(part 1 of 2)
# Autodesk Inventor assembly: Additional_Building
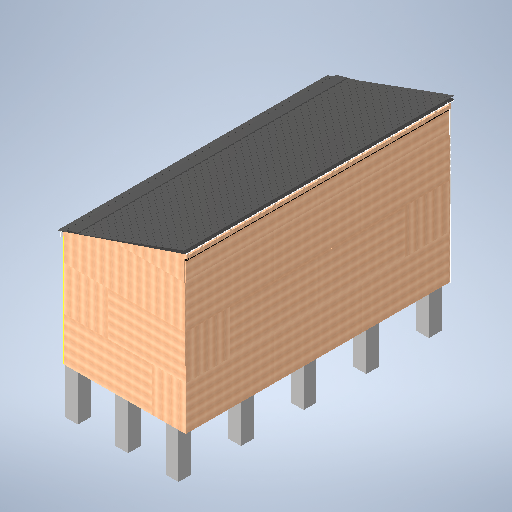
[picture p0: Inventor's stored thumbnail of the model, 512x512]
Saved by Autodesk Inventor 2025 (Build 290162010, 162A)
## iProperties
Created: 2024-08-02
Part Number: Additional_Building
Document SubType Name: Assembly
Designer: Tom
Author: Tom
## Documents named in this file (79)
- C:\Users\Tom\Documents\Inventor\Mobility\Additional_Building\Additional_Building.iam
- C:\Users\Tom\Documents\Inventor\Mobility\Additional_Building\Grid_Of_Piers.iam
- C:\Users\Tom\Documents\Inventor\Mobility\Additional_Building\Floor_System.iam
- C:\Users\Tom\Documents\Inventor\Mobility\Additional_Building\Framing_For_First_Floor.iam
- C:\Users\Tom\Documents\Inventor\Mobility\Additional_Building\Truss.iam
- C:\Users\Tom\Documents\Inventor\Mobility\Additional_Building\OSB_For_Walls_With_Dimensions_48_x_96_Inches.ipt
- C:\Users\Tom\Documents\Inventor\Mobility\Additional_Building\OSB_For_Walls_With_Dimensions_48_x_48_Inches.ipt
- C:\Users\Tom\Documents\Inventor\Mobility\Additional_Building\OSB_For_Roof_With_Dimensions_48_x_96.ipt
- C:\Users\Tom\Documents\Inventor\Mobility\Additional_Building\OSB_For_Walls_With_Dimensions_25.5_x_96_Inches.ipt
- C:\Users\Tom\Documents\Inventor\Mobility\Additional_Building\Subfascia_With_Dimensions_4.023_x_13.75_Inches.ipt
- C:\Users\Tom\Documents\Inventor\Mobility\Additional_Building\Subfascia_With_Dimensions_4.023_x_14.5_Inches.ipt
- C:\Users\Tom\Documents\Inventor\Mobility\Additional_Building\DensGlass_With_Dimensions_36.5_x_48_Inches.ipt
- C:\Users\Tom\Documents\Inventor\Mobility\Additional_Building\DensGlass_With_Dimensions_48_x_96_Inches.ipt
- C:\Users\Tom\Documents\Inventor\Mobility\Additional_Building\DensGlass_With_Dimensions_48_x_84.5_Inches.ipt
- C:\Users\Tom\Documents\Inventor\Mobility\Additional_Building\DensGlass_With_Dimensions_12_x_60.75_Inches.ipt
- C:\Users\Tom\Documents\Inventor\Mobility\Additional_Building\DensGlass_With_Dimensions_25.5_x_36.5_Inches.ipt
- C:\Users\Tom\Documents\Inventor\Mobility\Additional_Building\DensGlass_With_Dimensions_25.5_x_96_Inches.ipt
- C:\Users\Tom\Documents\Inventor\Mobility\Additional_Building\Siding_For_Back_Wall.iam
- C:\Users\Tom\Documents\Inventor\Mobility\Additional_Building\Fascia_For_Back.ipt
- C:\Users\Tom\Documents\Inventor\Mobility\Additional_Building\OSB_For_Side_And_Back.ipt
- C:\Users\Tom\Documents\Inventor\Mobility\Additional_Building\OSB_For_Roof_With_Dimensions_48_x_48.ipt
- C:\Users\Tom\Documents\Inventor\Mobility\Additional_Building\OSB_For_Roof_With_Dimensions_47.416_x_96.ipt
- C:\Users\Tom\Documents\Inventor\Mobility\Additional_Building\Stud_With_Height_4.254_Inches.ipt
- C:\Users\Tom\Documents\Inventor\Mobility\Additional_Building\Stud_With_Height_9.593_Inches.ipt
- C:\Users\Tom\Documents\Inventor\Mobility\Additional_Building\Stud_With_Height_14.931_Inches.ipt
- C:\Users\Tom\Documents\Inventor\Mobility\Additional_Building\Stud_With_Height_20.270_Inches.ipt
- C:\Users\Tom\Documents\Inventor\Mobility\Additional_Building\Stud_With_Height_25.608_Inches.ipt
- C:\Users\Tom\Documents\Inventor\Mobility\Additional_Building\Stud_With_Height_30.947_Inches.ipt
- C:\Users\Tom\Documents\Inventor\Mobility\Additional_Building\Stud_With_Height_36.285_Inches.ipt
- C:\Users\Tom\Documents\Inventor\Mobility\Additional_Building\Stud_With_Height_39.580_Inches.ipt
- C:\Users\Tom\Documents\Inventor\Mobility\Additional_Building\Stud_With_Height_41.707_Inches_And_Cut.ipt
- C:\Users\Tom\Documents\Inventor\Mobility\Additional_Building\Stud_With_Height_41.707_Inches.ipt
- C:\Users\Tom\Documents\Inventor\Mobility\Additional_Building\Support_For_Ceiling.ipt
- C:\Users\Tom\Documents\Inventor\Mobility\Additional_Building\OSB_For_Side_And_Front.ipt
- C:\Users\Tom\Documents\Inventor\Mobility\Additional_Building\OSB_For_Side_And_Top.ipt
- C:\Users\Tom\Documents\Inventor\Mobility\Additional_Building\Subfascia_With_Dimensions_3.725_x_13.75_Inches.ipt
- C:\Users\Tom\Documents\Inventor\Mobility\Additional_Building\Subfascia_With_Dimensions_3.725_x_14.5_Inches.ipt
- C:\Users\Tom\Documents\Inventor\Mobility\Additional_Building\OSB_For_Walls_With_Dimensions_21.107_x_48_Inches.ipt
- C:\Users\Tom\Documents\Inventor\Mobility\Additional_Building\OSB_For_Walls_With_Dimensions_21.107_x_96_Inches.ipt
- C:\Users\Tom\Documents\Inventor\Mobility\Additional_Building\Siding_For_Front_Wall.iam
- C:\Users\Tom\Documents\Inventor\Mobility\Additional_Building\Fascia_For_Front.ipt
- C:\Users\Tom\Documents\Inventor\Mobility\Additional_Building\OSB_For_Walls_With_Dimensions_48_x_85_Inches.ipt
- C:\Users\Tom\Documents\Inventor\Mobility\Additional_Building\OSB_For_Walls_With_Dimensions_37_x_48_Inches.ipt
- C:\Users\Tom\Documents\Inventor\Mobility\Additional_Building\Fascia_For_Side.ipt
- C:\Users\Tom\Documents\Inventor\Mobility\Additional_Building\Drip_Edge_For_Back.ipt
- C:\Users\Tom\Documents\Inventor\Mobility\Additional_Building\OSB_For_Rear_Roof.ipt
- C:\Users\Tom\Documents\Inventor\Mobility\Additional_Building\Siding_For_Left_Wall.iam
- C:\Users\Tom\Documents\Inventor\Mobility\Additional_Building\Siding_For_Right_Wall.iam
- C:\Users\Tom\Documents\Inventor\Mobility\Additional_Building\Drip_Edge_For_Side.ipt
- C:\Users\Tom\Documents\Inventor\Mobility\Additional_Building\Underlayment_For_Side.ipt
- C:\Users\Tom\Documents\Inventor\Mobility\Additional_Building\Underlayment_For_Front.ipt
- C:\Users\Tom\Documents\Inventor\Mobility\Additional_Building\Starter_Shingle_With_Dimensions_6.5_x_38_Inches.ipt
- C:\Users\Tom\Documents\Inventor\Mobility\Additional_Building\Leak_Barrier.ipt
- C:\Users\Tom\Documents\Inventor\Mobility\Additional_Building\Underlayment_For_Roof_With_Width_48_Inches.ipt
- C:\Users\Tom\Documents\Inventor\Mobility\Additional_Building\Underlayment_For_Roof_With_Width_19.157_Inches.ipt
- C:\Users\Tom\Documents\Inventor\Mobility\Additional_Building\Drip_Edge_For_Front.ipt
- C:\Users\Tom\Documents\Inventor\Mobility\Additional_Building\Starter_Shingle_With_Dimensions_6.5_x_35_Inches.ipt
- C:\Users\Tom\Documents\Inventor\Mobility\Additional_Building\Starter_Shingle_With_Dimensions_6.5_x_32.075_Inches.ipt
- C:\Users\Tom\Documents\Inventor\Mobility\Additional_Building\Starter_Shingle_With_Dimensions_6.5_x_29.875_Inches.ipt
- C:\Users\Tom\Documents\Inventor\Mobility\Additional_Building\Shingle_With_Dimensions_13.25_x_39.375_Inches.ipt
- C:\Users\Tom\Documents\Inventor\Mobility\Additional_Building\Shingle_With_Dimensions_13.25_x_19.45_Inches.ipt
- C:\Users\Tom\Documents\Inventor\Mobility\Additional_Building\Shingle_With_Dimensions_13.25_x_25.45_Inches.ipt
- C:\Users\Tom\Documents\Inventor\Mobility\Additional_Building\Bottom_Of_End_Cap_Of_Intake_Vent.ipt
- C:\Users\Tom\Documents\Inventor\Mobility\Additional_Building\Intake_Vent.ipt
- C:\Users\Tom\Documents\Inventor\Mobility\Additional_Building\Side_Of_End_Cap_For_Intake_Vent.ipt
- C:\Users\Tom\Documents\Inventor\Mobility\Additional_Building\First_Shingle_Over_Intake_Vent_With_Length_28.375_Inches.ipt
- C:\Users\Tom\Documents\Inventor\Mobility\Additional_Building\First_Shingle_Over_Intake_Vent_With_Length_39.375_Inches.ipt
- C:\Users\Tom\Documents\Inventor\Mobility\Additional_Building\First_Shingle_Over_Intake_Vent_With_Length_30.45_Inches.ipt
- C:\Users\Tom\Documents\Inventor\Mobility\Additional_Building\Second_Shingle_Over_Intake_Vent_With_Length_22.375_Inches.ipt
- C:\Users\Tom\Documents\Inventor\Mobility\Additional_Building\Second_Shingle_Over_Intake_Vent_With_Length_39.375_Inches.ipt
- C:\Users\Tom\Documents\Inventor\Mobility\Additional_Building\Second_Shingle_Over_Intake_Vent_With_Length_36.45_Inches.ipt
- C:\Users\Tom\Documents\Inventor\Mobility\Additional_Building\Third_Shingle_Over_Intake_Vent_With_Length_39.375_Inches.ipt
- C:\Users\Tom\Documents\Inventor\Mobility\Additional_Building\Third_Shingle_Over_Intake_Vent_With_Length_19.45_Inches.ipt
- C:\Users\Tom\Documents\Inventor\Mobility\Additional_Building\Shingle_With_Dimensions_13.25_x_33.375_Inches.ipt
- C:\Users\Tom\Documents\Inventor\Mobility\Additional_Building\Shingle_With_Dimensions_13.25_x_28.375_Inches.ipt
- C:\Users\Tom\Documents\Inventor\Mobility\Additional_Building\Shingle_With_Dimensions_13.25_x_30.45_Inches.ipt
- C:\Users\Tom\Documents\Inventor\Mobility\Additional_Building\Shingle_With_Dimensions_13.25_x_22.375_Inches.ipt
- C:\Users\Tom\Documents\Inventor\Mobility\Additional_Building\Shingle_With_Dimensions_13.25_x_36.45_Inches.ipt
- C:\Users\Tom\Documents\Inventor\Mobility\Additional_Building\Soffit_Strip_Vent.ipt
## Components (417 placed, 78 different names)
1. Grid_Of_Piers:1 [sub-assembly] — Mate:1, Flush:1, Mate:2
2. Floor_System:1 [sub-assembly] — Mate:1, Flush:1, Mate:2, Mate:3, Flush:2, Flush:3, Flush:15, Flush:16, Flush:29, Flush:30, Flush:31, Flush:33
3. Framing_For_First_Floor:1 [sub-assembly] — Mate:3, Flush:2, Flush:3, Flush:4, Flush:5, Mate:4, Flush:7, Mate:5, Mate:9, Mate:10, Flush:17, Mate:12, Mate:15, Mate:18, Mate:68, Flush:48, Flush:49, Mate:69, Flush:50, Flush:51, Mate:70, Flush:52, Flush:53, Mate:71, Flush:54, Flush:55, Mate:72, Flush:56, Flush:57, Mate:73, Flush:58, Flush:59, Mate:74, Flush:60, Flush:61, Mate:75, Flush:62, Flush:63, Mate:76, Flush:64, Mate:78, Mate:90, Mate:113, Mate:116, Mate:119, Mate:121
4. Subfascia_With_Dimensions_4.023_x_13.75_Inches:1 — Mate:21, Flush:22, Flush:23
5. Subfascia_With_Dimensions_4.023_x_13.75_Inches:2 — Flush:26, Mate:23, Flush:27, Flush:39
6. DensGlass_With_Dimensions_36.5_x_48_Inches:1 — Mate:24, Flush:28, Flush:29, Mate:26
7. DensGlass_With_Dimensions_36.5_x_48_Inches:2 — Mate:27, Mate:28, Flush:31
8. DensGlass_With_Dimensions_48_x_84.5_Inches:1 — Mate:29, Flush:32, Mate:30, Mate:32, Mate:38, Mate:41, Mate:44
9. DensGlass_With_Dimensions_48_x_96_Inches:3 — Mate:31, Mate:32, Mate:33, Mate:35
10. DensGlass_With_Dimensions_48_x_84.5_Inches:2 — Mate:34, Mate:35, Mate:36, Mate:47
11. DensGlass_With_Dimensions_25.5_x_36.5_Inches:1 — Mate:39, Mate:40, Mate:41, Mate:43
12. DensGlass_With_Dimensions_25.5_x_36.5_Inches:2 — Mate:45, Mate:46, Mate:47
13. Siding_For_Back_Wall:1 [sub-assembly] — Mate:48, Flush:34, Flush:35, Flush:158
14. Underlayment_For_Front:1 — Mate:146, Flush:126, Mate:147
15. Siding_For_Front_Wall:1 [sub-assembly] — Flush:93, Flush:94, Mate:108
16. Underlayment_For_Side:1 — Flush:122, Flush:157
17. Siding_For_Left_Wall:1 [sub-assembly] — Mate:133, Flush:117, Mate:134, Mate:207
18. Underlayment_For_Side:2 — Flush:124, Mate:145, Flush:125, Flush:126
19. Siding_For_Right_Wall:1 [sub-assembly] — Mate:135, Mate:136, Flush:118
20. Drip_Edge_For_Back:1 — Flush:109, Mate:128, Mate:137, Mate:188, Mate:189, Mate:202
21. Leak_Barrier:1 — Mate:188, Flush:153, Mate:189, Mate:190, Flush:154, Mate:191, Mate:199, Mate:210, Flush:180
22. Underlayment_For_Roof_With_Width_48_Inches:1 — Mate:190, Flush:154, Mate:191, Mate:192, Flush:155, Mate:193
23. Underlayment_For_Roof_With_Width_48_Inches:2 — Mate:192, Flush:155, Mate:193, Mate:194, Flush:156, Mate:195
24. Underlayment_For_Roof_With_Width_19.157_Inches:1 — Mate:194, Flush:156, Mate:195, Mate:198, Mate:209
25. Drip_Edge_For_Side:3 — Mate:197, Mate:198, Mate:199, Mate:211, Mate:213, Mate:214, Mate:215, Mate:216
26. Drip_Edge_For_Side:4 — Mate:208, Mate:209, Mate:210
27. Drip_Edge_For_Front:1 — Mate:211, Mate:212, Mate:213, Mate:223
28. Starter_Shingle_With_Dimensions_6.5_x_35_Inches:1 — Mate:214, Mate:215, Mate:216, Mate:218, Flush:159, Flush:160, Mate:222, Flush:163, Flush:164, Flush:172
29. Starter_Shingle_With_Dimensions_6.5_x_32.075_Inches:1 — Mate:220, Flush:161, Flush:162
30. Starter_Shingle_With_Dimensions_6.5_x_35_Inches:2 — Mate:225, Flush:166, Flush:167, Mate:226, Flush:168, Flush:169
31. Starter_Shingle_With_Dimensions_6.5_x_32.075_Inches:2 — Flush:170, Mate:227, Flush:171
32. Shingle_With_Dimensions_13.25_x_19.45_Inches:1 — Mate:229, Mate:230, Flush:174, Mate:232, Mate:264
33. Shingle_With_Dimensions_13.25_x_25.45_Inches:1 — Mate:232, Mate:234, Mate:240, Flush:185, Flush:186, Mate:263, Flush:203, Mate:264
34. Bottom_Of_End_Cap_Of_Intake_Vent:1 — Mate:234, Flush:179, Flush:180, Flush:181, Mate:235, Flush:182, Mate:237, Flush:183
35. Intake_Vent:1 — Flush:181, Mate:235, Flush:182, Mate:236, Mate:239, Mate:241, Mate:244
36. Side_Of_End_Cap_For_Intake_Vent:1 — Mate:236, Mate:237, Flush:183, Mate:238, Flush:184
37. Bottom_Of_End_Cap_Of_Intake_Vent:2 — Mate:238, Flush:184, Mate:239
38. Bottom_Of_End_Cap_Of_Intake_Vent:3 — Mate:240, Flush:185, Flush:186, Mate:242, Flush:187
39. Side_Of_End_Cap_For_Intake_Vent:2 — Mate:241, Mate:242, Flush:187, Mate:243, Flush:188
40. Bottom_Of_End_Cap_Of_Intake_Vent:4 — Mate:243, Mate:244, Flush:188
41. First_Shingle_Over_Intake_Vent_With_Length_28.375_Inches:1 — Mate:249, Flush:192, Mate:252, Flush:194, Flush:195, Flush:202, Flush:207
42. First_Shingle_Over_Intake_Vent_With_Length_30.45_Inches:1 — Mate:251, Flush:193, Mate:255, Flush:197
43. Second_Shingle_Over_Intake_Vent_With_Length_22.375_Inches:1 — Mate:252, Flush:194, Flush:195, Mate:254, Flush:196, Mate:257, Flush:198, Flush:199, Flush:201, Flush:207
44. Second_Shingle_Over_Intake_Vent_With_Length_36.45_Inches:1 — Mate:255, Flush:197, Mate:256, Mate:258
45. Third_Shingle_Over_Intake_Vent_With_Length_19.45_Inches:1 — Mate:258, Flush:200, Mate:259, Mate:269
46. Shingle_With_Dimensions_13.25_x_39.375_Inches:8 — Flush:205, Mate:267, Flush:206
47. Shingle_With_Dimensions_13.25_x_33.375_Inches:1 — Mate:265, Mate:266, Mate:268, Flush:208, Mate:271, Flush:210, Flush:211
48. Shingle_With_Dimensions_13.25_x_25.45_Inches:2 — Mate:269, Mate:270, Flush:209, Mate:274, Flush:214
49. Shingle_With_Dimensions_13.25_x_28.375_Inches:1 — Mate:271, Flush:210, Flush:211, Mate:273, Flush:212, Mate:275, Flush:215, Flush:216
50. Shingle_With_Dimensions_13.25_x_30.45_Inches:1 — Mate:274, Flush:213, Flush:214, Mate:278
51. Shingle_With_Dimensions_13.25_x_22.375_Inches:1 — Mate:275, Flush:215, Flush:216, Mate:277, Flush:217, Mate:280, Flush:219, Flush:220
52. Shingle_With_Dimensions_13.25_x_36.45_Inches:1 — Mate:278, Mate:279, Flush:218, Mate:281
53. Shingle_With_Dimensions_13.25_x_19.45_Inches:2 — Mate:281, Mate:282, Flush:221, Mate:286
54. Shingle_With_Dimensions_13.25_x_33.375_Inches:2 — Mate:283, Flush:222, Flush:223, Mate:285, Flush:224, Mate:288, Flush:226, Flush:227
55. Shingle_With_Dimensions_13.25_x_25.45_Inches:3 — Mate:286, Mate:287, Flush:225, Mate:291
56. Shingle_With_Dimensions_13.25_x_28.375_Inches:2 — Mate:288, Flush:226, Flush:227, Mate:290, Flush:228, Mate:293, Flush:230, Flush:231
57. Shingle_With_Dimensions_13.25_x_30.45_Inches:2 — Mate:291, Mate:292, Flush:229, Mate:296
58. Shingle_With_Dimensions_13.25_x_22.375_Inches:2 — Mate:293, Flush:230, Flush:231, Mate:295, Flush:232, Mate:298, Flush:234, Flush:235
59. Shingle_With_Dimensions_13.25_x_36.45_Inches:2 — Mate:296, Mate:297, Flush:233, Mate:299
60. Shingle_With_Dimensions_13.25_x_19.45_Inches:3 — Mate:299, Mate:300, Flush:236, Mate:304
61. Shingle_With_Dimensions_13.25_x_33.375_Inches:3 — Mate:301, Flush:237, Flush:238, Mate:303, Flush:239, Mate:306, Flush:241, Flush:242
62. Shingle_With_Dimensions_13.25_x_25.45_Inches:4 — Mate:304, Mate:305, Flush:240, Mate:309
63. Shingle_With_Dimensions_13.25_x_28.375_Inches:3 — Mate:306, Flush:241, Flush:242, Mate:308, Flush:243, Mate:311, Flush:245, Flush:246
64. Shingle_With_Dimensions_13.25_x_30.45_Inches:3 — Mate:309, Mate:310, Flush:244, Mate:314
65. Shingle_With_Dimensions_13.25_x_22.375_Inches:3 — Mate:311, Flush:245, Flush:246, Mate:313, Flush:247, Mate:316, Flush:249, Flush:250
66. Shingle_With_Dimensions_13.25_x_36.45_Inches:3 — Mate:314, Mate:315, Flush:248, Mate:317
67. Shingle_With_Dimensions_13.25_x_19.45_Inches:4 — Mate:317, Mate:318, Flush:251, Mate:322
68. Shingle_With_Dimensions_13.25_x_33.375_Inches:4 — Mate:319, Flush:252, Flush:253, Mate:321, Flush:254, Mate:324, Flush:256, Flush:257
69. Shingle_With_Dimensions_13.25_x_25.45_Inches:5 — Mate:322, Mate:323, Flush:255, Mate:327
70. Shingle_With_Dimensions_13.25_x_28.375_Inches:4 — Mate:324, Flush:256, Flush:257, Mate:326, Flush:258, Mate:329, Flush:260, Flush:261
71. Shingle_With_Dimensions_13.25_x_30.45_Inches:4 — Mate:327, Mate:328, Flush:259, Mate:332
72. Shingle_With_Dimensions_13.25_x_22.375_Inches:4 — Mate:329, Flush:260, Flush:261, Mate:331, Flush:262, Mate:334, Flush:264, Flush:265
73. Shingle_With_Dimensions_13.25_x_36.45_Inches:4 — Mate:332, Mate:333, Flush:263, Mate:335
74. Shingle_With_Dimensions_13.25_x_19.45_Inches:5 — Mate:335, Mate:336, Flush:266, Mate:340
75. Shingle_With_Dimensions_13.25_x_33.375_Inches:5 — Mate:337, Flush:267, Flush:268, Mate:339, Flush:269, Mate:342, Flush:271, Flush:272
76. Shingle_With_Dimensions_13.25_x_25.45_Inches:6 — Mate:340, Mate:341, Flush:270, Mate:345
77. Shingle_With_Dimensions_13.25_x_28.375_Inches:5 — Mate:342, Flush:271, Flush:272, Mate:344, Flush:273, Mate:347, Flush:275, Flush:276
78. Shingle_With_Dimensions_13.25_x_30.45_Inches:5 — Mate:345, Mate:346, Flush:274, Mate:350
79. Shingle_With_Dimensions_13.25_x_36.45_Inches:5 — Mate:350, Mate:351, Flush:278, Mate:353
80. Shingle_With_Dimensions_13.25_x_22.375_Inches:5 — Mate:347, Flush:275, Flush:276, Mate:349, Flush:277, Mate:352, Flush:279, Flush:280
81. Shingle_With_Dimensions_13.25_x_19.45_Inches:6 — Mate:353, Mate:354, Flush:281
82. Soffit_Strip_Vent:1 — Flush:282, Flush:283, Flush:284
83. Truss:1 [sub-assembly] — Flush:6, Mate:23, Flush:27, Mate:50, Mate:56, Mate:77, Mate:79, Flush:65, Flush:67, Flush:69, Flush:71, Flush:73, Flush:75, Flush:77, Flush:79, Flush:81, Mate:92, Mate:109, Flush:104, Flush:115, Mate:132, Flush:116, Mate:153, Mate:184, Flush:151
84. Truss:2 [sub-assembly] — Flush:4, Flush:5, Mate:4, Mate:20, Mate:101, Flush:91, Mate:103, Flush:92, Flush:124, Mate:147, Flush:127
85. Truss:3 [sub-assembly] — Flush:6, Flush:7, Mate:5, Flush:26, Mate:81, Mate:82, Mate:83, Mate:84, Mate:85, Mate:86, Mate:87, Mate:88, Mate:89, Mate:91, Flush:82, Mate:99, Flush:87, Flush:88
86. Truss:4 [sub-assembly] — Mate:100, Flush:89, Flush:90
87. Truss:5 [sub-assembly]
88. Truss:6 [sub-assembly]
89. Truss:7 [sub-assembly]
90. Truss:8 [sub-assembly]
91. Truss:9 [sub-assembly]
92. Truss:10 [sub-assembly]
93. Truss:11 [sub-assembly]
94. Truss:12 [sub-assembly]
95. Truss:13 [sub-assembly]
96. Truss:14 [sub-assembly]
97. Truss:15 [sub-assembly] — Mate:63
98. Truss:16 [sub-assembly] — Mate:105
99. Truss:17 [sub-assembly]
100. Truss:18 [sub-assembly] — Mate:22, Flush:25
101. Truss:19 [sub-assembly] — Mate:21, Flush:22, Flush:23, Flush:24, Mate:149
102. OSB_For_Walls_With_Dimensions_25.5_x_96_Inches:1 — Mate:18, Flush:18, Mate:20, Mate:39
103. OSB_For_Walls_With_Dimensions_25.5_x_96_Inches:2 — Mate:42
104. OSB_For_Walls_With_Dimensions_25.5_x_96_Inches:3 — Mate:45
105. OSB_For_Walls_With_Dimensions_48_x_48_Inches:2 — Mate:15, Mate:16, Mate:17, Mate:29, Flush:32
106. OSB_For_Walls_With_Dimensions_48_x_48_Inches:1 — Mate:10, Mate:11, Flush:17, Mate:13, Mate:34
107. OSB_For_Walls_With_Dimensions_48_x_48_Inches:3 — Mate:102
108. OSB_For_Walls_With_Dimensions_48_x_48_Inches:4
109. OSB_For_Walls_With_Dimensions_48_x_96_Inches:13 — Mate:101, Mate:102, Flush:91, Mate:104, Mate:108
110. OSB_For_Walls_With_Dimensions_48_x_96_Inches:14 — Mate:106
111. OSB_For_Walls_With_Dimensions_48_x_96_Inches:15 — Mate:146
112. OSB_For_Walls_With_Dimensions_21.107_x_96_Inches:1 — Mate:105, Mate:106, Mate:107
113. OSB_For_Walls_With_Dimensions_21.107_x_96_Inches:2
114. OSB_For_Walls_With_Dimensions_21.107_x_48_Inches:1 — Mate:103, Mate:104, Flush:92, Mate:107
115. OSB_For_Walls_With_Dimensions_21.107_x_48_Inches:2
116. Subfascia_With_Dimensions_4.023_x_14.5_Inches:1 — Flush:24, Mate:22, Flush:25
117. Subfascia_With_Dimensions_4.023_x_14.5_Inches:2
118. Subfascia_With_Dimensions_4.023_x_14.5_Inches:3
119. Subfascia_With_Dimensions_4.023_x_14.5_Inches:4
120. Subfascia_With_Dimensions_4.023_x_14.5_Inches:5
121. Subfascia_With_Dimensions_4.023_x_14.5_Inches:6
122. Subfascia_With_Dimensions_4.023_x_14.5_Inches:7
123. Subfascia_With_Dimensions_4.023_x_14.5_Inches:8
124. Subfascia_With_Dimensions_4.023_x_14.5_Inches:9
125. Subfascia_With_Dimensions_4.023_x_14.5_Inches:10
126. Subfascia_With_Dimensions_4.023_x_14.5_Inches:11
127. Subfascia_With_Dimensions_4.023_x_14.5_Inches:12
128. Subfascia_With_Dimensions_4.023_x_14.5_Inches:13
129. Subfascia_With_Dimensions_4.023_x_14.5_Inches:14
130. Subfascia_With_Dimensions_4.023_x_14.5_Inches:15
131. Subfascia_With_Dimensions_4.023_x_14.5_Inches:16
132. DensGlass_With_Dimensions_48_x_96_Inches:1 — Mate:25, Mate:26, Flush:30, Mate:30, Mate:33
133. DensGlass_With_Dimensions_48_x_96_Inches:2 — Mate:28, Mate:36
134. DensGlass_With_Dimensions_12_x_60.75_Inches:1 — Mate:37, Mate:38, Flush:33
135. DensGlass_With_Dimensions_12_x_60.75_Inches:2 — Mate:48, Flush:34, Flush:35, Flush:158
136. DensGlass_With_Dimensions_12_x_60.75_Inches:3 — Mate:40
137. DensGlass_With_Dimensions_12_x_60.75_Inches:4 — Mate:57, Mate:115, Flush:157
138. DensGlass_With_Dimensions_25.5_x_96_Inches:1 — Mate:42, Mate:43, Mate:44
139. DensGlass_With_Dimensions_25.5_x_96_Inches:2 — Mate:46
140. Stud_With_Height_4.254_Inches:1 — Mate:68, Flush:48, Flush:49, Flush:66
141. Stud_With_Height_9.593_Inches:1 — Mate:69, Flush:50, Flush:51, Flush:68
142. Stud_With_Height_14.931_Inches:1 — Mate:70, Flush:52, Flush:53, Flush:70
143. Stud_With_Height_20.270_Inches:1 — Mate:71, Flush:54, Flush:55, Flush:72
144. Stud_With_Height_25.608_Inches:1 — Mate:72, Flush:56, Flush:57, Flush:74
145. Stud_With_Height_30.947_Inches:1 — Mate:73, Flush:58, Flush:59, Flush:76
146. Stud_With_Height_36.285_Inches:1 — Mate:74, Flush:60, Flush:61, Flush:78
147. Stud_With_Height_41.707_Inches_And_Cut:1 — Mate:76, Mate:77, Flush:64, Mate:80
148. Stud_With_Height_39.580_Inches:1 — Mate:75, Flush:62, Flush:63, Flush:80
149. Stud_With_Height_4.254_Inches:2
150. Stud_With_Height_9.593_Inches:2
151. Stud_With_Height_14.931_Inches:2
152. Stud_With_Height_20.270_Inches:2
153. Stud_With_Height_25.608_Inches:2
154. Stud_With_Height_30.947_Inches:2
155. Stud_With_Height_36.285_Inches:2
156. Stud_With_Height_41.707_Inches_And_Cut:2
157. Stud_With_Height_39.580_Inches:2
158. Stud_With_Height_41.707_Inches:1 — Mate:78, Mate:79, Mate:80
159. Stud_With_Height_41.707_Inches:2
160. Support_For_Ceiling:9 — Mate:89, Flush:81, Mate:90
161. Support_For_Ceiling:1 — Mate:81, Flush:65, Flush:66
162. Support_For_Ceiling:2 — Mate:82, Flush:67, Flush:68
163. Support_For_Ceiling:3 — Mate:83, Flush:69, Flush:70
164. Support_For_Ceiling:4 — Mate:84, Flush:71, Flush:72
165. Support_For_Ceiling:5 — Mate:85, Flush:73, Flush:74
166. Support_For_Ceiling:6 — Mate:86, Flush:75, Flush:76
167. Support_For_Ceiling:7 — Mate:87, Flush:77, Flush:78
168. Support_For_Ceiling:8 — Mate:88, Flush:79, Flush:80
169. Support_For_Ceiling:10 — Mate:91, Flush:82, Mate:92
170. Support_For_Ceiling:11
171. Support_For_Ceiling:12
172. Support_For_Ceiling:13
173. Support_For_Ceiling:14
174. Support_For_Ceiling:15
175. Support_For_Ceiling:16
176. Support_For_Ceiling:17
177. Support_For_Ceiling:18
178. Support_For_Ceiling:19
179. Support_For_Ceiling:20
180. Subfascia_With_Dimensions_3.725_x_13.75_Inches:1 — Mate:99, Flush:87, Flush:88
181. Subfascia_With_Dimensions_3.725_x_13.75_Inches:2
182. Subfascia_With_Dimensions_3.725_x_14.5_Inches:1 — Mate:100, Flush:89, Flush:90
183. Subfascia_With_Dimensions_3.725_x_14.5_Inches:2
184. Subfascia_With_Dimensions_3.725_x_14.5_Inches:3
185. Subfascia_With_Dimensions_3.725_x_14.5_Inches:4
186. Subfascia_With_Dimensions_3.725_x_14.5_Inches:5
187. Subfascia_With_Dimensions_3.725_x_14.5_Inches:6
188. Subfascia_With_Dimensions_3.725_x_14.5_Inches:7
189. Subfascia_With_Dimensions_3.725_x_14.5_Inches:8
190. Subfascia_With_Dimensions_3.725_x_14.5_Inches:9
191. Subfascia_With_Dimensions_3.725_x_14.5_Inches:10
192. Subfascia_With_Dimensions_3.725_x_14.5_Inches:11
193. Subfascia_With_Dimensions_3.725_x_14.5_Inches:12
194. Subfascia_With_Dimensions_3.725_x_14.5_Inches:13
195. Subfascia_With_Dimensions_3.725_x_14.5_Inches:14
196. Subfascia_With_Dimensions_3.725_x_14.5_Inches:15
197. Subfascia_With_Dimensions_3.725_x_14.5_Inches:16
198. Fascia_For_Back:1 — Mate:50, Flush:39, Flush:104, Flush:105, Flush:109, Mate:128, Mate:134
199. Fascia_For_Back:2
200. Fascia_For_Back:3 — Mate:136
201. Fascia_For_Front:1 — Mate:109, Mate:126, Mate:186, Mate:207, Mate:212, Flush:282, Flush:283, Flush:284
202. Fascia_For_Front:2
203. Fascia_For_Front:3
204. OSB_For_Walls_With_Dimensions_48_x_96_Inches:16 — Mate:119, Mate:120, Flush:98, Mate:131, Mate:133, Flush:117
205. OSB_For_Walls_With_Dimensions_37_x_48_Inches:1 — Mate:121, Mate:122, Mate:131, Flush:122
206. OSB_For_Walls_With_Dimensions_48_x_48_Inches:5 — Mate:113, Mate:114, Mate:115, Mate:117, Mate:120
207. OSB_For_Walls_With_Dimensions_48_x_85_Inches:1 — Mate:116, Mate:117, Mate:118, Mate:122
208. OSB_For_Side_And_Back:1 — Mate:56, Mate:57, Flush:83, Mate:98, Mate:111, Mate:112, Mate:114, Mate:118, Flush:128, Mate:185
209. OSB_For_Side_And_Front:1 — Flush:83, Mate:111, Mate:112, Mate:355
210. OSB_For_Side_And_Top:1 — Mate:184, Mate:185, Flush:151, Mate:355
211. OSB_For_Walls_With_Dimensions_48_x_96_Inches:17 — Mate:135
212. OSB_For_Walls_With_Dimensions_37_x_48_Inches:2 — Flush:118
213. OSB_For_Walls_With_Dimensions_48_x_48_Inches:6
214. OSB_For_Walls_With_Dimensions_48_x_85_Inches:2
215. OSB_For_Side_And_Back:2
216. OSB_For_Side_And_Front:2
217. OSB_For_Side_And_Top:2 — Mate:145, Mate:148
218. OSB_For_Rear_Roof:1 — Flush:115, Mate:132, Flush:116, Flush:128
219. OSB_For_Rear_Roof:2 — Mate:137
220. OSB_For_Rear_Roof:3 — Mate:150, Mate:151
221. OSB_For_Roof_With_Dimensions_48_x_48:1 — Mate:65, Mate:148, Mate:149, Mate:150, Mate:152
222. OSB_For_Roof_With_Dimensions_48_x_48:2
223. OSB_For_Roof_With_Dimensions_48_x_96:4 — Mate:63, Mate:65, Mate:151
224. OSB_For_Roof_With_Dimensions_48_x_96:5
225. OSB_For_Roof_With_Dimensions_47.416_x_96:1 — Mate:152, Mate:153, Flush:127
226. OSB_For_Roof_With_Dimensions_47.416_x_96:2
227. OSB_For_Roof_With_Dimensions_47.416_x_96:3 — Mate:186
228. Fascia_For_Side:1 — Mate:126, Flush:105, Mate:187, Flush:153, Mate:197, Mate:202
229. Fascia_For_Side:2 — Mate:208
230. Starter_Shingle_With_Dimensions_6.5_x_38_Inches:19 — Mate:218, Flush:159, Flush:160
231. Starter_Shingle_With_Dimensions_6.5_x_38_Inches:20
232. Starter_Shingle_With_Dimensions_6.5_x_38_Inches:21
233. Starter_Shingle_With_Dimensions_6.5_x_38_Inches:22
234. Starter_Shingle_With_Dimensions_6.5_x_38_Inches:23
235. Starter_Shingle_With_Dimensions_6.5_x_38_Inches:24 — Mate:220, Flush:161, Flush:162
236. Starter_Shingle_With_Dimensions_6.5_x_29.875_Inches:1 — Mate:223, Mate:224, Flush:165, Mate:225, Flush:166, Flush:167
237. Starter_Shingle_With_Dimensions_6.5_x_29.875_Inches:2
238. Starter_Shingle_With_Dimensions_6.5_x_38_Inches:31 — Mate:226, Flush:168, Flush:169
239. Starter_Shingle_With_Dimensions_6.5_x_38_Inches:32
240. Starter_Shingle_With_Dimensions_6.5_x_38_Inches:33
241. Starter_Shingle_With_Dimensions_6.5_x_38_Inches:34
242. Starter_Shingle_With_Dimensions_6.5_x_38_Inches:35
243. Starter_Shingle_With_Dimensions_6.5_x_38_Inches:36 — Flush:170, Mate:227, Flush:171
244. Shingle_With_Dimensions_13.25_x_39.375_Inches:1 — Mate:228, Flush:172, Flush:173, Flush:175, Mate:231, Flush:202
245. Shingle_With_Dimensions_13.25_x_39.375_Inches:2
246. Shingle_With_Dimensions_13.25_x_39.375_Inches:3
247. Shingle_With_Dimensions_13.25_x_39.375_Inches:4
248. Shingle_With_Dimensions_13.25_x_39.375_Inches:5
249. Shingle_With_Dimensions_13.25_x_39.375_Inches:6
250. Shingle_With_Dimensions_13.25_x_39.375_Inches:7 — Mate:230, Flush:174
251. Shingle_With_Dimensions_13.25_x_39.375_Inches:14 — Flush:175, Flush:176, Mate:231, Flush:179
252. Shingle_With_Dimensions_13.25_x_39.375_Inches:15
253. Shingle_With_Dimensions_13.25_x_39.375_Inches:16
254. Shingle_With_Dimensions_13.25_x_39.375_Inches:17
255. Shingle_With_Dimensions_13.25_x_39.375_Inches:18
256. Shingle_With_Dimensions_13.25_x_39.375_Inches:19
257. Shingle_With_Dimensions_13.25_x_39.375_Inches:20 — Mate:263, Flush:203
258. First_Shingle_Over_Intake_Vent_With_Length_39.375_Inches:1 — Mate:249, Flush:192, Mate:253
259. First_Shingle_Over_Intake_Vent_With_Length_39.375_Inches:2
260. First_Shingle_Over_Intake_Vent_With_Length_39.375_Inches:3
261. First_Shingle_Over_Intake_Vent_With_Length_39.375_Inches:4
262. First_Shingle_Over_Intake_Vent_With_Length_39.375_Inches:5
263. First_Shingle_Over_Intake_Vent_With_Length_39.375_Inches:6 — Mate:251, Flush:193
264. Second_Shingle_Over_Intake_Vent_With_Length_39.375_Inches:1 — Mate:253, Mate:254, Flush:196
265. Second_Shingle_Over_Intake_Vent_With_Length_39.375_Inches:2
266. Second_Shingle_Over_Intake_Vent_With_Length_39.375_Inches:3
267. Second_Shingle_Over_Intake_Vent_With_Length_39.375_Inches:4
268. Second_Shingle_Over_Intake_Vent_With_Length_39.375_Inches:5
269. Second_Shingle_Over_Intake_Vent_With_Length_39.375_Inches:6 — Mate:256
270. Third_Shingle_Over_Intake_Vent_With_Length_39.375_Inches:1 — Mate:257, Flush:198, Flush:199, Flush:201, Flush:205, Mate:265, Mate:266, Flush:206
271. Third_Shingle_Over_Intake_Vent_With_Length_39.375_Inches:2
272. Third_Shingle_Over_Intake_Vent_With_Length_39.375_Inches:3
273. Third_Shingle_Over_Intake_Vent_With_Length_39.375_Inches:4
274. Third_Shingle_Over_Intake_Vent_With_Length_39.375_Inches:5
275. Third_Shingle_Over_Intake_Vent_With_Length_39.375_Inches:6
276. Third_Shingle_Over_Intake_Vent_With_Length_39.375_Inches:7 — Flush:200, Mate:259
277. Shingle_With_Dimensions_13.25_x_39.375_Inches:21 — Mate:267, Mate:268, Flush:208, Mate:272
278. Shingle_With_Dimensions_13.25_x_39.375_Inches:22
279. Shingle_With_Dimensions_13.25_x_39.375_Inches:23
280. Shingle_With_Dimensions_13.25_x_39.375_Inches:24
281. Shingle_With_Dimensions_13.25_x_39.375_Inches:25
282. Shingle_With_Dimensions_13.25_x_39.375_Inches:26 — Mate:270, Flush:209
283. Shingle_With_Dimensions_13.25_x_39.375_Inches:27 — Mate:272, Mate:273, Flush:212, Mate:276
284. Shingle_With_Dimensions_13.25_x_39.375_Inches:28
285. Shingle_With_Dimensions_13.25_x_39.375_Inches:29
286. Shingle_With_Dimensions_13.25_x_39.375_Inches:30
287. Shingle_With_Dimensions_13.25_x_39.375_Inches:31
288. Shingle_With_Dimensions_13.25_x_39.375_Inches:32 — Flush:213
289. Shingle_With_Dimensions_13.25_x_39.375_Inches:33 — Mate:276, Mate:277, Flush:217
290. Shingle_With_Dimensions_13.25_x_39.375_Inches:34
291. Shingle_With_Dimensions_13.25_x_39.375_Inches:35
292. Shingle_With_Dimensions_13.25_x_39.375_Inches:36
293. Shingle_With_Dimensions_13.25_x_39.375_Inches:37
294. Shingle_With_Dimensions_13.25_x_39.375_Inches:38 — Mate:279, Flush:218
295. Shingle_With_Dimensions_13.25_x_39.375_Inches:39 — Mate:280, Flush:219, Flush:220, Mate:283, Flush:222, Flush:223
296. Shingle_With_Dimensions_13.25_x_39.375_Inches:40 — Mate:284
297. Shingle_With_Dimensions_13.25_x_39.375_Inches:41
298. Shingle_With_Dimensions_13.25_x_39.375_Inches:42
299. Shingle_With_Dimensions_13.25_x_39.375_Inches:43
300. Shingle_With_Dimensions_13.25_x_39.375_Inches:44
301. Shingle_With_Dimensions_13.25_x_39.375_Inches:45 — Mate:282, Flush:221
302. Shingle_With_Dimensions_13.25_x_39.375_Inches:46 — Mate:284, Mate:285, Flush:224, Mate:289
303. Shingle_With_Dimensions_13.25_x_39.375_Inches:47
304. Shingle_With_Dimensions_13.25_x_39.375_Inches:48
305. Shingle_With_Dimensions_13.25_x_39.375_Inches:49
306. Shingle_With_Dimensions_13.25_x_39.375_Inches:50
307. Shingle_With_Dimensions_13.25_x_39.375_Inches:51 — Mate:287, Flush:225
308. Shingle_With_Dimensions_13.25_x_39.375_Inches:52 — Mate:289, Mate:290, Flush:228, Mate:294
309. Shingle_With_Dimensions_13.25_x_39.375_Inches:53
310. Shingle_With_Dimensions_13.25_x_39.375_Inches:54
311. Shingle_With_Dimensions_13.25_x_39.375_Inches:55
312. Shingle_With_Dimensions_13.25_x_39.375_Inches:56
313. Shingle_With_Dimensions_13.25_x_39.375_Inches:57 — Mate:292, Flush:229
314. Shingle_With_Dimensions_13.25_x_39.375_Inches:58 — Mate:294, Mate:295, Flush:232
315. Shingle_With_Dimensions_13.25_x_39.375_Inches:59
316. Shingle_With_Dimensions_13.25_x_39.375_Inches:60
317. Shingle_With_Dimensions_13.25_x_39.375_Inches:61
318. Shingle_With_Dimensions_13.25_x_39.375_Inches:62
319. Shingle_With_Dimensions_13.25_x_39.375_Inches:63 — Mate:297, Flush:233
320. Shingle_With_Dimensions_13.25_x_39.375_Inches:64 — Mate:298, Flush:234, Flush:235, Mate:301, Flush:237, Flush:238
321. Shingle_With_Dimensions_13.25_x_39.375_Inches:65 — Mate:302
322. Shingle_With_Dimensions_13.25_x_39.375_Inches:66
323. Shingle_With_Dimensions_13.25_x_39.375_Inches:67
324. Shingle_With_Dimensions_13.25_x_39.375_Inches:68
325. Shingle_With_Dimensions_13.25_x_39.375_Inches:69
326. Shingle_With_Dimensions_13.25_x_39.375_Inches:70 — Mate:300, Flush:236
327. Shingle_With_Dimensions_13.25_x_39.375_Inches:71 — Mate:302, Mate:303, Flush:239, Mate:307
328. Shingle_With_Dimensions_13.25_x_39.375_Inches:72
329. Shingle_With_Dimensions_13.25_x_39.375_Inches:73
330. Shingle_With_Dimensions_13.25_x_39.375_Inches:74
331. Shingle_With_Dimensions_13.25_x_39.375_Inches:75
332. Shingle_With_Dimensions_13.25_x_39.375_Inches:76 — Mate:305, Flush:240
333. Shingle_With_Dimensions_13.25_x_39.375_Inches:77 — Mate:307, Mate:308, Flush:243, Mate:312
334. Shingle_With_Dimensions_13.25_x_39.375_Inches:78
335. Shingle_With_Dimensions_13.25_x_39.375_Inches:79
336. Shingle_With_Dimensions_13.25_x_39.375_Inches:80
337. Shingle_With_Dimensions_13.25_x_39.375_Inches:81
338. Shingle_With_Dimensions_13.25_x_39.375_Inches:82 — Mate:310, Flush:244
339. Shingle_With_Dimensions_13.25_x_39.375_Inches:83 — Mate:312, Mate:313, Flush:247
340. Shingle_With_Dimensions_13.25_x_39.375_Inches:84
341. Shingle_With_Dimensions_13.25_x_39.375_Inches:85
342. Shingle_With_Dimensions_13.25_x_39.375_Inches:86
343. Shingle_With_Dimensions_13.25_x_39.375_Inches:87
344. Shingle_With_Dimensions_13.25_x_39.375_Inches:88 — Mate:315, Flush:248
345. Shingle_With_Dimensions_13.25_x_39.375_Inches:89 — Mate:316, Flush:249, Flush:250, Mate:319, Flush:252, Flush:253
346. Shingle_With_Dimensions_13.25_x_39.375_Inches:90 — Mate:320
347. Shingle_With_Dimensions_13.25_x_39.375_Inches:91
348. Shingle_With_Dimensions_13.25_x_39.375_Inches:92
349. Shingle_With_Dimensions_13.25_x_39.375_Inches:93
350. Shingle_With_Dimensions_13.25_x_39.375_Inches:94
351. Shingle_With_Dimensions_13.25_x_39.375_Inches:95 — Mate:318, Flush:251
352. Shingle_With_Dimensions_13.25_x_39.375_Inches:96 — Mate:320, Mate:321, Flush:254, Mate:325
353. Shingle_With_Dimensions_13.25_x_39.375_Inches:97
354. Shingle_With_Dimensions_13.25_x_39.375_Inches:98
355. Shingle_With_Dimensions_13.25_x_39.375_Inches:99
356. Shingle_With_Dimensions_13.25_x_39.375_Inches:100
357. Shingle_With_Dimensions_13.25_x_39.375_Inches:101 — Mate:323, Flush:255
358. Shingle_With_Dimensions_13.25_x_39.375_Inches:102 — Mate:325, Mate:326, Flush:258, Mate:330
359. Shingle_With_Dimensions_13.25_x_39.375_Inches:103
360. Shingle_With_Dimensions_13.25_x_39.375_Inches:104
361. Shingle_With_Dimensions_13.25_x_39.375_Inches:105
362. Shingle_With_Dimensions_13.25_x_39.375_Inches:106
363. Shingle_With_Dimensions_13.25_x_39.375_Inches:107 — Mate:328, Flush:259
364. Shingle_With_Dimensions_13.25_x_39.375_Inches:108 — Mate:330, Mate:331, Flush:262
365. Shingle_With_Dimensions_13.25_x_39.375_Inches:109
366. Shingle_With_Dimensions_13.25_x_39.375_Inches:110
367. Shingle_With_Dimensions_13.25_x_39.375_Inches:111
368. Shingle_With_Dimensions_13.25_x_39.375_Inches:112
369. Shingle_With_Dimensions_13.25_x_39.375_Inches:113 — Mate:333, Flush:263
370. Shingle_With_Dimensions_13.25_x_39.375_Inches:114 — Mate:334, Flush:264, Flush:265, Mate:337, Flush:267, Flush:268
371. Shingle_With_Dimensions_13.25_x_39.375_Inches:115 — Mate:338
372. Shingle_With_Dimensions_13.25_x_39.375_Inches:116
373. Shingle_With_Dimensions_13.25_x_39.375_Inches:117
374. Shingle_With_Dimensions_13.25_x_39.375_Inches:118
375. Shingle_With_Dimensions_13.25_x_39.375_Inches:119
376. Shingle_With_Dimensions_13.25_x_39.375_Inches:120 — Mate:336, Flush:266
377. Shingle_With_Dimensions_13.25_x_39.375_Inches:121 — Mate:338, Mate:339, Flush:269, Mate:343
378. Shingle_With_Dimensions_13.25_x_39.375_Inches:122
379. Shingle_With_Dimensions_13.25_x_39.375_Inches:123
380. Shingle_With_Dimensions_13.25_x_39.375_Inches:124
381. Shingle_With_Dimensions_13.25_x_39.375_Inches:125
382. Shingle_With_Dimensions_13.25_x_39.375_Inches:126 — Mate:341, Flush:270
383. Shingle_With_Dimensions_13.25_x_39.375_Inches:127 — Mate:343, Mate:344, Flush:273, Mate:348
384. Shingle_With_Dimensions_13.25_x_39.375_Inches:128
385. Shingle_With_Dimensions_13.25_x_39.375_Inches:129
386. Shingle_With_Dimensions_13.25_x_39.375_Inches:130
387. Shingle_With_Dimensions_13.25_x_39.375_Inches:131
388. Shingle_With_Dimensions_13.25_x_39.375_Inches:132 — Mate:346, Flush:274
389. Shingle_With_Dimensions_13.25_x_39.375_Inches:133 — Mate:348, Mate:349, Flush:277
390. Shingle_With_Dimensions_13.25_x_39.375_Inches:134
391. Shingle_With_Dimensions_13.25_x_39.375_Inches:135
392. Shingle_With_Dimensions_13.25_x_39.375_Inches:136
393. Shingle_With_Dimensions_13.25_x_39.375_Inches:137
394. Shingle_With_Dimensions_13.25_x_39.375_Inches:138 — Mate:351, Flush:278
395. Shingle_With_Dimensions_13.25_x_39.375_Inches:139 — Mate:352, Flush:279, Flush:280
396. Shingle_With_Dimensions_13.25_x_39.375_Inches:140
397. Shingle_With_Dimensions_13.25_x_39.375_Inches:141
398. Shingle_With_Dimensions_13.25_x_39.375_Inches:142
399. Shingle_With_Dimensions_13.25_x_39.375_Inches:143
400. Shingle_With_Dimensions_13.25_x_39.375_Inches:144
401. Shingle_With_Dimensions_13.25_x_39.375_Inches:145 — Mate:354, Flush:281
402. OSB_For_Walls_With_Dimensions_48_x_96_Inches:1 — Mate:9, Flush:15, Flush:16, Mate:11, Mate:16, Flush:18, Mate:24, Flush:28, Mate:25, Mate:37
403. OSB_For_Walls_With_Dimensions_48_x_96_Inches:2
404. OSB_For_Walls_With_Dimensions_48_x_96_Inches:3 — Mate:14, Mate:27, Flush:98
405. OSB_For_Walls_With_Dimensions_48_x_96_Inches:4 — Mate:12, Mate:13, Mate:14, Mate:31
406. OSB_For_Walls_With_Dimensions_48_x_96_Inches:5 — Mate:17
407. OSB_For_Walls_With_Dimensions_48_x_96_Inches:8 — Flush:93, Flush:94, Flush:125
408. OSB_For_Walls_With_Dimensions_48_x_96_Inches:9
409. OSB_For_Walls_With_Dimensions_48_x_96_Inches:10
410. OSB_For_Walls_With_Dimensions_48_x_96_Inches:11
411. OSB_For_Walls_With_Dimensions_48_x_96_Inches:12
412. Starter_Shingle_With_Dimensions_6.5_x_38_Inches:25 — Mate:222, Flush:163, Flush:164, Mate:228, Flush:173, Flush:176
413. Starter_Shingle_With_Dimensions_6.5_x_38_Inches:26
414. Starter_Shingle_With_Dimensions_6.5_x_38_Inches:27 — Mate:224, Flush:165
415. Starter_Shingle_With_Dimensions_6.5_x_38_Inches:28 — Mate:229
416. Starter_Shingle_With_Dimensions_6.5_x_38_Inches:29
417. Starter_Shingle_With_Dimensions_6.5_x_38_Inches:30
## Component patterns: (2 elements, first: Truss:1), (17 elements, first: Truss:3), (3 elements, first: OSB_For_Walls_With_Dimensions_25.5_x_96_Inches:1), (2 elements, first: OSB_For_Walls_With_Dimensions_48_x_48_Inches:2 + OSB_For_Walls_With_Dimensions_48_x_48_Inches:1), (3 elements, first: OSB_For_Walls_With_Dimensions_48_x_96_Inches:13), (2 elements, first: OSB_For_Walls_With_Dimensions_21.107_x_96_Inches:1), (2 elements, first: OSB_For_Walls_With_Dimensions_21.107_x_48_Inches:1), (16 elements, first: Subfascia_With_Dimensions_4.023_x_14.5_Inches:1), (2 elements, first: DensGlass_With_Dimensions_48_x_96_Inches:1), (4 elements, first: DensGlass_With_Dimensions_12_x_60.75_Inches:1), (2 elements, first: DensGlass_With_Dimensions_25.5_x_96_Inches:1), (2 elements, first: Stud_With_Height_4.254_Inches:1 + Stud_With_Height_9.593_Inches:1 + Stud_With_Height_14.931_Inches:1 + Stud_With_Height_20.270_Inches:1 + Stud_With_Height_25.608_Inches:1 + Stud_With_Height_30.947_Inches:1 + Stud_With_Height_36.285_Inches:1 + Stud_With_Height_41.707_Inches_And_Cut:1 + Stud_With_Height_39.580_Inches:1), (2 elements, first: Stud_With_Height_41.707_Inches:1), (2 elements, first: Support_For_Ceiling:9 + Support_For_Ceiling:1 + Support_For_Ceiling:2 + Support_For_Ceiling:3 + Support_For_Ceiling:4 + Support_For_Ceiling:5 + Support_For_Ceiling:6 + Support_For_Ceiling:7 + Support_For_Ceiling:8 + Support_For_Ceiling:10), (2 elements, first: Subfascia_With_Dimensions_3.725_x_13.75_Inches:1), (16 elements, first: Subfascia_With_Dimensions_3.725_x_14.5_Inches:1), (3 elements, first: Fascia_For_Back:1), (3 elements, first: Fascia_For_Front:1), (2 elements, first: OSB_For_Walls_With_Dimensions_48_x_96_Inches:16 + OSB_For_Walls_With_Dimensions_37_x_48_Inches:1 + OSB_For_Walls_With_Dimensions_48_x_48_Inches:5 + OSB_For_Walls_With_Dimensions_48_x_85_Inches:1 + OSB_For_Side_And_Back:1 + OSB_For_Side_And_Front:1 + OSB_For_Side_And_Top:1), (3 elements, first: OSB_For_Rear_Roof:1), (2 elements, first: OSB_For_Roof_With_Dimensions_48_x_48:1), (2 elements, first: OSB_For_Roof_With_Dimensions_48_x_96:4), (3 elements, first: OSB_For_Roof_With_Dimensions_47.416_x_96:1), (2 elements, first: Fascia_For_Side:1), (6 elements, first: Starter_Shingle_With_Dimensions_6.5_x_38_Inches:19), (2 elements, first: Starter_Shingle_With_Dimensions_6.5_x_29.875_Inches:1), (6 elements, first: Starter_Shingle_With_Dimensions_6.5_x_38_Inches:31), (7 elements, first: Shingle_With_Dimensions_13.25_x_39.375_Inches:1), (7 elements, first: Shingle_With_Dimensions_13.25_x_39.375_Inches:14), (6 elements, first: First_Shingle_Over_Intake_Vent_With_Length_39.375_Inches:1), (6 elements, first: Second_Shingle_Over_Intake_Vent_With_Length_39.375_Inches:1), (7 elements, first: Third_Shingle_Over_Intake_Vent_With_Length_39.375_Inches:1), (6 elements, first: Shingle_With_Dimensions_13.25_x_39.375_Inches:21), (6 elements, first: Shingle_With_Dimensions_13.25_x_39.375_Inches:27), (6 elements, first: Shingle_With_Dimensions_13.25_x_39.375_Inches:33), (7 elements, first: Shingle_With_Dimensions_13.25_x_39.375_Inches:39), (6 elements, first: Shingle_With_Dimensions_13.25_x_39.375_Inches:46), (6 elements, first: Shingle_With_Dimensions_13.25_x_39.375_Inches:52), (6 elements, first: Shingle_With_Dimensions_13.25_x_39.375_Inches:58), (7 elements, first: Shingle_With_Dimensions_13.25_x_39.375_Inches:64), (6 elements, first: Shingle_With_Dimensions_13.25_x_39.375_Inches:71), (6 elements, first: Shingle_With_Dimensions_13.25_x_39.375_Inches:77), (6 elements, first: Shingle_With_Dimensions_13.25_x_39.375_Inches:83), (7 elements, first: Shingle_With_Dimensions_13.25_x_39.375_Inches:89), (6 elements, first: Shingle_With_Dimensions_13.25_x_39.375_Inches:96), (6 elements, first: Shingle_With_Dimensions_13.25_x_39.375_Inches:102), (6 elements, first: Shingle_With_Dimensions_13.25_x_39.375_Inches:108), (7 elements, first: Shingle_With_Dimensions_13.25_x_39.375_Inches:114), (6 elements, first: Shingle_With_Dimensions_13.25_x_39.375_Inches:121), (6 elements, first: Shingle_With_Dimensions_13.25_x_39.375_Inches:127), (6 elements, first: Shingle_With_Dimensions_13.25_x_39.375_Inches:133), (7 elements, first: Shingle_With_Dimensions_13.25_x_39.375_Inches:139), (3 elements, first: OSB_For_Walls_With_Dimensions_48_x_96_Inches:1), (2 elements, first: OSB_For_Walls_With_Dimensions_48_x_96_Inches:4), Component Pattern 3:2 (3 elements), Component Pattern 4:2 (2 elements), (3 elements, first: Starter_Shingle_With_Dimensions_6.5_x_38_Inches:25), Component Pattern 41:2 (3 elements)
## Relationships (482: Mate 269, Flush 211, Angle 2)
- Mate:1: Grid_Of_Piers:1 ↔ Floor_System:1
- Flush:1: Grid_Of_Piers:1 ↔ Floor_System:1
- Mate:2: Grid_Of_Piers:1 ↔ Floor_System:1
- Mate:3: Floor_System:1 ↔ Framing_For_First_Floor:1
- Flush:2: Floor_System:1 ↔ Framing_For_First_Floor:1
- Flush:3: Floor_System:1 ↔ Framing_For_First_Floor:1
- Flush:4: Framing_For_First_Floor:1 ↔ Truss:2
- Flush:5: Framing_For_First_Floor:1 ↔ Truss:2
- Mate:4: Framing_For_First_Floor:1 ↔ Truss:2
- Flush:6 (387.35 mm): Truss:1 ↔ Truss:3
- Flush:7: Framing_For_First_Floor:1 ↔ Truss:3
- Mate:5: Framing_For_First_Floor:1 ↔ Truss:3
- Mate:9: Framing_For_First_Floor:1 ↔ OSB_For_Walls_With_Dimensions_48_x_96_Inches:1
- Flush:15: Floor_System:1 ↔ OSB_For_Walls_With_Dimensions_48_x_96_Inches:1
- Flush:16: Floor_System:1 ↔ OSB_For_Walls_With_Dimensions_48_x_96_Inches:1
- Mate:10: Framing_For_First_Floor:1 ↔ OSB_For_Walls_With_Dimensions_48_x_48_Inches:1
- Mate:11: OSB_For_Walls_With_Dimensions_48_x_48_Inches:1 ↔ OSB_For_Walls_With_Dimensions_48_x_96_Inches:1
- Flush:17: Framing_For_First_Floor:1 ↔ OSB_For_Walls_With_Dimensions_48_x_48_Inches:1
- Mate:12: Framing_For_First_Floor:1 ↔ OSB_For_Walls_With_Dimensions_48_x_96_Inches:4
- Mate:13: OSB_For_Walls_With_Dimensions_48_x_48_Inches:1 ↔ OSB_For_Walls_With_Dimensions_48_x_96_Inches:4
- Mate:14: OSB_For_Walls_With_Dimensions_48_x_96_Inches:3 ↔ OSB_For_Walls_With_Dimensions_48_x_96_Inches:4
- Mate:15: Framing_For_First_Floor:1 ↔ OSB_For_Walls_With_Dimensions_48_x_48_Inches:2
- Mate:16: OSB_For_Walls_With_Dimensions_48_x_48_Inches:2 ↔ OSB_For_Walls_With_Dimensions_48_x_96_Inches:1
- Mate:17: OSB_For_Walls_With_Dimensions_48_x_48_Inches:2 ↔ OSB_For_Walls_With_Dimensions_48_x_96_Inches:5
- Mate:18: Framing_For_First_Floor:1 ↔ OSB_For_Walls_With_Dimensions_25.5_x_96_Inches:1
- Flush:18: OSB_For_Walls_With_Dimensions_25.5_x_96_Inches:1 ↔ OSB_For_Walls_With_Dimensions_48_x_96_Inches:1
- Mate:20: Truss:2 ↔ OSB_For_Walls_With_Dimensions_25.5_x_96_Inches:1
- Mate:21: Subfascia_With_Dimensions_4.023_x_13.75_Inches:1 ↔ Truss:19
- Flush:22: Subfascia_With_Dimensions_4.023_x_13.75_Inches:1 ↔ Truss:19
- Flush:23: Subfascia_With_Dimensions_4.023_x_13.75_Inches:1 ↔ Truss:19
- Flush:24: Truss:19 ↔ Subfascia_With_Dimensions_4.023_x_14.5_Inches:1
- Mate:22: Truss:18 ↔ Subfascia_With_Dimensions_4.023_x_14.5_Inches:1
- Flush:25: Truss:18 ↔ Subfascia_With_Dimensions_4.023_x_14.5_Inches:1
- Flush:26: Subfascia_With_Dimensions_4.023_x_13.75_Inches:2 ↔ Truss:3
- Mate:23: Subfascia_With_Dimensions_4.023_x_13.75_Inches:2 ↔ Truss:1
- Flush:27: Subfascia_With_Dimensions_4.023_x_13.75_Inches:2 ↔ Truss:1
- Mate:24: DensGlass_With_Dimensions_36.5_x_48_Inches:1 ↔ OSB_For_Walls_With_Dimensions_48_x_96_Inches:1
- Flush:28 (292.1 mm): DensGlass_With_Dimensions_36.5_x_48_Inches:1 ↔ OSB_For_Walls_With_Dimensions_48_x_96_Inches:1
- Flush:29: Floor_System:1 ↔ DensGlass_With_Dimensions_36.5_x_48_Inches:1
- Mate:25: DensGlass_With_Dimensions_48_x_96_Inches:1 ↔ OSB_For_Walls_With_Dimensions_48_x_96_Inches:1
- Mate:26: DensGlass_With_Dimensions_36.5_x_48_Inches:1 ↔ DensGlass_With_Dimensions_48_x_96_Inches:1
- Flush:30: Floor_System:1 ↔ DensGlass_With_Dimensions_48_x_96_Inches:1
- Mate:27: DensGlass_With_Dimensions_36.5_x_48_Inches:2 ↔ OSB_For_Walls_With_Dimensions_48_x_96_Inches:3
- Mate:28: DensGlass_With_Dimensions_36.5_x_48_Inches:2 ↔ DensGlass_With_Dimensions_48_x_96_Inches:2
- Flush:31: Floor_System:1 ↔ DensGlass_With_Dimensions_36.5_x_48_Inches:2
- Mate:29: DensGlass_With_Dimensions_48_x_84.5_Inches:1 ↔ OSB_For_Walls_With_Dimensions_48_x_48_Inches:2
- Flush:32 (292.1 mm): DensGlass_With_Dimensions_48_x_84.5_Inches:1 ↔ OSB_For_Walls_With_Dimensions_48_x_48_Inches:2
- Mate:30: DensGlass_With_Dimensions_48_x_84.5_Inches:1 ↔ DensGlass_With_Dimensions_48_x_96_Inches:1
- Mate:31: DensGlass_With_Dimensions_48_x_96_Inches:3 ↔ OSB_For_Walls_With_Dimensions_48_x_96_Inches:4
- Mate:32: DensGlass_With_Dimensions_48_x_84.5_Inches:1 ↔ DensGlass_With_Dimensions_48_x_96_Inches:3
- Mate:33: DensGlass_With_Dimensions_48_x_96_Inches:3 ↔ DensGlass_With_Dimensions_48_x_96_Inches:1
- Mate:34: DensGlass_With_Dimensions_48_x_84.5_Inches:2 ↔ OSB_For_Walls_With_Dimensions_48_x_48_Inches:1
- Mate:35: DensGlass_With_Dimensions_48_x_96_Inches:3 ↔ DensGlass_With_Dimensions_48_x_84.5_Inches:2
- Mate:36: DensGlass_With_Dimensions_48_x_84.5_Inches:2 ↔ DensGlass_With_Dimensions_48_x_96_Inches:2
- Mate:37: DensGlass_With_Dimensions_12_x_60.75_Inches:1 ↔ OSB_For_Walls_With_Dimensions_48_x_96_Inches:1
- Mate:38: DensGlass_With_Dimensions_48_x_84.5_Inches:1 ↔ DensGlass_With_Dimensions_12_x_60.75_Inches:1
- Flush:33: Floor_System:1 ↔ DensGlass_With_Dimensions_12_x_60.75_Inches:1
- Mate:39: DensGlass_With_Dimensions_25.5_x_36.5_Inches:1 ↔ OSB_For_Walls_With_Dimensions_25.5_x_96_Inches:1
- Mate:40: DensGlass_With_Dimensions_25.5_x_36.5_Inches:1 ↔ DensGlass_With_Dimensions_12_x_60.75_Inches:3
- Mate:41: DensGlass_With_Dimensions_48_x_84.5_Inches:1 ↔ DensGlass_With_Dimensions_25.5_x_36.5_Inches:1
- Mate:42: OSB_For_Walls_With_Dimensions_25.5_x_96_Inches:2 ↔ DensGlass_With_Dimensions_25.5_x_96_Inches:1
- Mate:43: DensGlass_With_Dimensions_25.5_x_36.5_Inches:1 ↔ DensGlass_With_Dimensions_25.5_x_96_Inches:1
- Mate:44: DensGlass_With_Dimensions_48_x_84.5_Inches:1 ↔ DensGlass_With_Dimensions_25.5_x_96_Inches:1
- Mate:45: DensGlass_With_Dimensions_25.5_x_36.5_Inches:2 ↔ OSB_For_Walls_With_Dimensions_25.5_x_96_Inches:3
- Mate:46: DensGlass_With_Dimensions_25.5_x_36.5_Inches:2 ↔ DensGlass_With_Dimensions_25.5_x_96_Inches:2
- Mate:47: DensGlass_With_Dimensions_48_x_84.5_Inches:2 ↔ DensGlass_With_Dimensions_25.5_x_36.5_Inches:2
- Mate:48: Siding_For_Back_Wall:1 ↔ DensGlass_With_Dimensions_12_x_60.75_Inches:2
- Flush:34: Siding_For_Back_Wall:1 ↔ DensGlass_With_Dimensions_12_x_60.75_Inches:2
- Flush:35: Siding_For_Back_Wall:1 ↔ DensGlass_With_Dimensions_12_x_60.75_Inches:2
- Mate:50: Truss:1 ↔ Fascia_For_Back:1
- Flush:39 (-29.3688 mm): Subfascia_With_Dimensions_4.023_x_13.75_Inches:2 ↔ Fascia_For_Back:1
- Mate:56: Truss:1 ↔ OSB_For_Side_And_Back:1
- Mate:57: DensGlass_With_Dimensions_12_x_60.75_Inches:4 ↔ OSB_For_Side_And_Back:1
- Mate:63: Truss:15 ↔ OSB_For_Roof_With_Dimensions_48_x_96:4
- Mate:65: OSB_For_Roof_With_Dimensions_48_x_48:1 ↔ OSB_For_Roof_With_Dimensions_48_x_96:4
- Mate:68: Framing_For_First_Floor:1 ↔ Stud_With_Height_4.254_Inches:1
- Flush:48: Framing_For_First_Floor:1 ↔ Stud_With_Height_4.254_Inches:1
- Flush:49: Framing_For_First_Floor:1 ↔ Stud_With_Height_4.254_Inches:1